# Autodesk Inventor assembly: gearbox
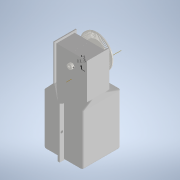
[picture p0: Inventor's stored thumbnail of the model, 180x180]
Saved by Autodesk Inventor 2020 (Build 240168000, 168)
## iProperties
Created: 2019-06-21
Part Number: gearbox
Document SubType Name: Assembly
Designer: User
Author: User
## Documents named in this file (10)
- F:\Library\Documents\Project_quick_temp\Gear_box_3\gearbox.iam
- F:\Library\Documents\Project_quick_temp\Gear_box_3\gearbox\设计加速器\锥齿轮1.iam
- F:\Library\Documents\Project_quick_temp\Gear_box_3\gearbox\设计加速器\正齿轮1.iam
- F:\Library\Documents\Project_quick_temp\Gear_box_3\gearbox\设计加速器\正齿轮2.iam
- F:\Library\Documents\Project_quick_temp\Gear_box_3\gearbox\设计加速器\正齿轮3.iam
- F:\Library\Documents\Project_quick_temp\Gear_box_3\gearbox\设计加速器\正齿轮4.iam
- F:\Library\Documents\Project_quick_temp\Gear_box_3\Base_Bottom.ipt
- F:\Library\Documents\Project_quick_temp\Gear_box_3\Base_Top.ipt
- F:\Library\Documents\Project_quick_temp\Gear_box_3\gearbox\设计加速器\螺栓联接1.iam
- F:\Library\Documents\Project_quick_temp\Gear_box_3\gearbox\设计加速器\螺栓联接2.iam
## Components (9 placed, 5 different names)
1. 锥齿轮:1 [sub-assembly] — 表面齐平:1, 配合:1, 配合:2, 配合:3, 配合:4, 配合:5, 配合:9, 配合:11, 配合:13, 表面齐平:3
2. 正齿轮:1 [sub-assembly] — 配合:1, 配合:2, 配合:3, 配合:6, 配合:12
3. 正齿轮:2 [sub-assembly] — 配合:4, 配合:5, 配合:6, 配合:7, 配合:8
4. 正齿轮:3 [sub-assembly] — 配合:7, 配合:8, 配合:9, 配合:10
5. 正齿轮:4 [sub-assembly] — 配合:10, 配合:11, 配合:12, 配合:13, 表面齐平:2
6. Base_Bottom:1 — 表面齐平:4
7. Base_Top:1 — 表面齐平:5, 配合:14, 配合:15, 配合:16, 配合:17
8. 螺栓联接:1 [sub-assembly] — 配合:14, 配合:15
9. 螺栓联接:2 [sub-assembly] — 配合:16, 配合:17
## Relationships (22: Mate 17, Flush 5)
- 表面齐平:1 [Flush] (-2.5 mm): 锥齿轮:1
- 配合:1 [Mate]: 锥齿轮:1 ↔ 正齿轮:1
- 配合:2 [Mate]: 锥齿轮:1 ↔ 正齿轮:1
- 配合:3 [Mate]: 锥齿轮:1 ↔ 正齿轮:1
- 配合:4 [Mate]: 锥齿轮:1 ↔ 正齿轮:2
- 配合:5 [Mate]: 锥齿轮:1 ↔ 正齿轮:2
- 配合:6 [Mate]: 正齿轮:1 ↔ 正齿轮:2
- 配合:7 [Mate]: 正齿轮:2 ↔ 正齿轮:3
- 配合:8 [Mate]: 正齿轮:2 ↔ 正齿轮:3
- 配合:9 [Mate]: 锥齿轮:1 ↔ 正齿轮:3
- 配合:10 [Mate]: 正齿轮:3 ↔ 正齿轮:4
- 配合:11 [Mate]: 锥齿轮:1 ↔ 正齿轮:4
- 配合:12 [Mate]: 正齿轮:1 ↔ 正齿轮:4
- 配合:13 [Mate]: 锥齿轮:1 ↔ 正齿轮:4
- 表面齐平:2 [Flush] (-1.5 mm): 正齿轮:4
- 表面齐平:3 [Flush] (50 mm): 锥齿轮:1
- 表面齐平:4 [Flush]: Base_Bottom:1
- 表面齐平:5 [Flush]: Base_Top:1
- 配合:14 [Mate]: Base_Top:1 ↔ 螺栓联接:1
- 配合:15 [Mate]: Base_Top:1 ↔ 螺栓联接:1
- 配合:16 [Mate]: Base_Top:1 ↔ 螺栓联接:2
- 配合:17 [Mate]: Base_Top:1 ↔ 螺栓联接:2
